# Autodesk Inventor assembly: plateaumonte6GV2202
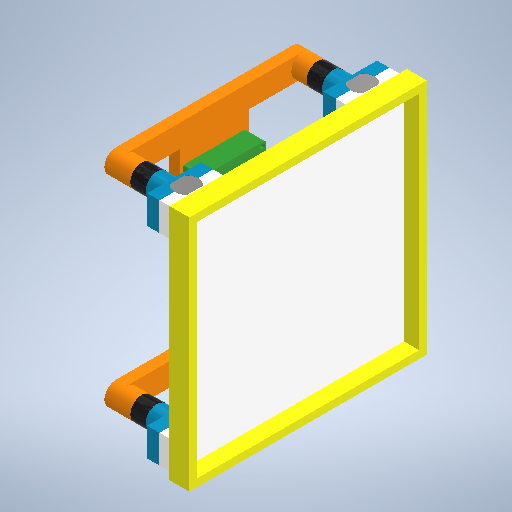
[picture p0: Inventor's stored thumbnail of the model, 512x512]
Saved by Autodesk Inventor 2025.2 (Build 292293000, 293)
## iProperties
Created: 2025-02-21
Part Number: plateaumonte6GV2202
Document SubType Name: Assembly
Designer: antoi
Author: antoi
## Documents named in this file (10)
- C:\Users\antoi\Documents\Henallux_24_25\Q2\proj\prototype\plateaumonte6GV2202.iam
- C:\Users\antoi\Documents\Henallux_24_25\Q2\proj\prototype\moteurG6V2.ipt
- C:\Users\antoi\Documents\Henallux_24_25\Q2\proj\prototype\plateauV2102.ipt
- C:\Users\antoi\Documents\Henallux_24_25\Q2\proj\prototype\bagueSilentbloc.ipt
- C:\Users\antoi\Documents\Henallux_24_25\Q2\proj\prototype\rebord1515.ipt
- C:\Users\antoi\Documents\Henallux_24_25\Q2\proj\prototype\silentBloc.ipt
- C:\Users\antoi\Documents\Henallux_24_25\Q2\proj\prototype\MPU6050.ipt
- C:\Users\antoi\Documents\Henallux_24_25\Q2\proj\prototype\MPU6050_MIR1.ipt
- C:\Users\antoi\Documents\Henallux_24_25\Q2\proj\prototype\MDD3A.ipt
- C:\Users\antoi\Documents\Henallux_24_25\Q2\proj\prototype\base.ipt
## Components (21 placed, 9 different names)
1. plateauV2102:1 — Placage:1, Affleurement:1, Affleurement:2, Affleurement:3, Placage:3, Placage:4, Placage:5, Placage:8, Placage:9, Placage:10
2. rebord1515:1 — Placage:3, Placage:4, Placage:5
3. MPU6050_MIR1:1
4. MPU6050_MIR1:2
5. MDD3A:1 — Placage:11, Placage:12, Placage:13
6. base:1 — Placage:11, Placage:12, Placage:13, Placage:14, Placage:15, Placage:16, Placage:17, Placage:18, Placage:19
7. MDD3A:2 — Placage:14, Placage:15, Placage:16
8. moteurG6V2:1 — Placage:1, Affleurement:1
9. moteurG6V2:2 — Placage:2
10. moteurG6V2:3
11. moteurG6V2:4
12. bagueSilentbloc:1 — Placage:2, Affleurement:2, Affleurement:3
13. bagueSilentbloc:2 — Placage:6, Placage:7
14. bagueSilentbloc:3
15. bagueSilentbloc:4
16. silentBloc:1 — Placage:6, Placage:7, Placage:19
17. silentBloc:2 — Placage:17
18. silentBloc:3
19. silentBloc:4 — Placage:18
20. MPU6050:1 — Placage:8, Placage:9, Placage:10
21. MPU6050:2
## Component patterns: (4 elements, first: moteurG6V2:1), (4 elements, first: bagueSilentbloc:1), (4 elements, first: silentBloc:1), (2 elements, first: MPU6050:1)
## Relationships (22: Mate 19, Flush 3)
- Placage:1 [Mate]: plateauV2102:1 ↔ moteurG6V2:1
- Affleurement:1 [Flush]: plateauV2102:1 ↔ moteurG6V2:1
- Placage:2 [Mate]: moteurG6V2:2 ↔ bagueSilentbloc:1
- Affleurement:2 [Flush]: plateauV2102:1 ↔ bagueSilentbloc:1
- Affleurement:3 [Flush]: plateauV2102:1 ↔ bagueSilentbloc:1
- Placage:3 [Mate]: plateauV2102:1 ↔ rebord1515:1
- Placage:4 [Mate]: plateauV2102:1 ↔ rebord1515:1
- Placage:5 [Mate]: plateauV2102:1 ↔ rebord1515:1
- Placage:6 [Mate]: bagueSilentbloc:2 ↔ silentBloc:1
- Placage:7 [Mate]: bagueSilentbloc:2 ↔ silentBloc:1
- Placage:8 [Mate]: plateauV2102:1 ↔ MPU6050:1
- Placage:9 [Mate]: plateauV2102:1 ↔ MPU6050:1
- Placage:10 [Mate]: plateauV2102:1 ↔ MPU6050:1
- Placage:11 [Mate]: MDD3A:1 ↔ base:1
- Placage:12 [Mate]: MDD3A:1 ↔ base:1
- Placage:13 [Mate]: MDD3A:1 ↔ base:1
- Placage:14 [Mate]: base:1 ↔ MDD3A:2
- Placage:15 [Mate]: base:1 ↔ MDD3A:2
- Placage:16 [Mate]: base:1 ↔ MDD3A:2
- Placage:17 [Mate]: base:1 ↔ silentBloc:2
- Placage:18 [Mate]: base:1 ↔ silentBloc:4
- Placage:19 [Mate]: base:1 ↔ silentBloc:1
